# Autodesk Inventor assembly: 4xStack
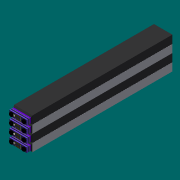
[picture p0: Inventor's stored thumbnail of the model, 180x180]
Saved by Autodesk Inventor 2016 SP1 (Build 200210100, 210)
## iProperties
Created: 2016-02-15
Part Number: 4xStack
Document SubType Name: Assembly
Designer: sawai
Author: sawai
## Documents named in this file (3)
- C:\Users\sawai\OneDrive\projects\scintillatorPanel\4xStack.iam
- C:\Users\sawai\OneDrive\projects\scintillatorPanel\scintillatorPanel.iam
- C:\Users\sawai\OneDrive\projects\scintillatorPanel\coluredSpacer.ipt
## Components (6 placed, 2 different names)
1. scintillatorPanel:1 [sub-assembly] — Flush:3, Flush:6, Mate:1, Mate:5, Mate:8
2. scintillatorPanel:2 [sub-assembly] — Flush:2, Flush:3, Flush:5, Flush:6, Mate:1, Mate:2, Mate:9
3. scintillatorPanel:3 [sub-assembly] — Flush:1, Flush:2, Flush:4, Flush:5, Mate:2, Mate:3, Mate:4, Mate:6
4. scintillatorPanel:4 [sub-assembly] — Flush:1, Flush:4, Mate:3, Mate:7
5. coluredSpacer:1 — Mate:5, Mate:8, Mate:9
6. coluredSpacer:2 — Mate:4, Mate:6, Mate:7
## Relationships (15: Mate 9, Flush 6)
- Flush:1: scintillatorPanel:3 ↔ scintillatorPanel:4
- Flush:2: scintillatorPanel:2 ↔ scintillatorPanel:3
- Flush:3: scintillatorPanel:1 ↔ scintillatorPanel:2
- Flush:4: scintillatorPanel:3 ↔ scintillatorPanel:4
- Flush:5: scintillatorPanel:2 ↔ scintillatorPanel:3
- Flush:6: scintillatorPanel:1 ↔ scintillatorPanel:2
- Mate:1: scintillatorPanel:1 ↔ scintillatorPanel:2
- Mate:2: scintillatorPanel:2 ↔ scintillatorPanel:3
- Mate:3: scintillatorPanel:3 ↔ scintillatorPanel:4
- Mate:4: scintillatorPanel:3 ↔ coluredSpacer:2
- Mate:5: scintillatorPanel:1 ↔ coluredSpacer:1
- Mate:6: scintillatorPanel:3 ↔ coluredSpacer:2
- Mate:7: scintillatorPanel:4 ↔ coluredSpacer:2
- Mate:8: scintillatorPanel:1 ↔ coluredSpacer:1
- Mate:9: scintillatorPanel:2 ↔ coluredSpacer:1
